# Autodesk Inventor assembly: rotation_sensor_tracking_wheel
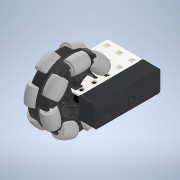
[picture p0: Inventor's stored thumbnail of the model, 180x180]
Saved by Autodesk Inventor 2022 (Build 260153000, 153)
## iProperties
Created: 2021-11-26
Part Number: rotation_sensor_tracking_wheel
Document SubType Name: Assembly
Designer: Alex
Author: Alex
## Documents named in this file (4)
- C:\Users\Alex\Documents\robotics\cad\DecBot\333B\tracking_wheels\rotation_sensor_tracking_wheel.iam
- C:\Users\Alex\Documents\robotics\cad\Library 1.2\Structure\C-Channels\Aluminum 1x3x1\1x3x1x5 Aluminum.ipt
- C:\Users\Alex\Documents\robotics\cad\Library 1.2\Motion\Wheels\Omnis\2.75 Omni - New, Square.ipt
- C:\Users\Alex\Documents\robotics\cad\Library 1.2\Electronics\Sensors\V5 Rotation Sensor.ipt
## Components (3 placed, 3 different names)
1. 1x3x1x5 Aluminum:1 — Insert:1, Insert:2
2. 2.75 Omni - New, Square:1 — Insert:1
3. V5 Rotation Sensor:1 — Insert:2
## Relationships (2: Insert 2)
- Insert:1 (6.35 mm): 1x3x1x5 Aluminum:1 ↔ 2.75 Omni - New, Square:1
- Insert:2: 1x3x1x5 Aluminum:1 ↔ V5 Rotation Sensor:1
